# Autodesk Inventor assembly: Skateboard Remote
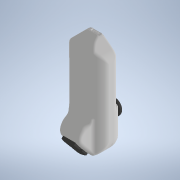
[picture p0: Inventor's stored thumbnail of the model, 180x180]
Saved by Autodesk Inventor 2020 (Build 240168000, 168)
## iProperties
Created: 2021-01-14
Part Number: Skateboard Remote
Document SubType Name: Assembly
Designer: Luke
Author: Luke
## Documents named in this file (19)
- C:\Users\Luke\Documents\Git Projects\Electric Skateboard V2\Part Files\Remote Parts\Skateboard Remote.iam
- C:\Users\Luke\Documents\Git Projects\Electric Skateboard V2\Part Files\Remote Parts\PCB.ipt
- C:\Users\Luke\Documents\Git Projects\Electric Skateboard V2\Part Files\Remote Parts\Battery Spacer.ipt
- C:\Users\Luke\Documents\Git Projects\Electric Skateboard V2\Part Files\Remote Parts\Battery.ipt
- C:\Users\Luke\Documents\Git Projects\Electric Skateboard V2\Part Files\Remote Parts\Button Module.ipt
- C:\Users\Luke\Documents\Git Projects\Electric Skateboard V2\Part Files\Remote Parts\Joystick.ipt
- C:\Users\Luke\Documents\Git Projects\Electric Skateboard V2\Part Files\Remote Parts\Button.ipt
- C:\Users\Luke\Documents\Git Projects\Electric Skateboard V2\Part Files\Remote Parts\Joystick Cap.ipt
- C:\Users\Luke\Documents\Git Projects\Electric Skateboard V2\Part Files\Remote Parts\Display.ipt
- C:\Users\Luke\Documents\Git Projects\Electric Skateboard V2\Part Files\Remote Parts\Vibrator Motor.ipt
- C:\Users\Luke\Documents\Git Projects\Electric Skateboard V2\Part Files\Remote Parts\USB Port.ipt
- C:\Users\Luke\Documents\Git Projects\Electric Skateboard V2\Part Files\Remote Parts\BMS.ipt
- C:\Users\Luke\Documents\Git Projects\Electric Skateboard V2\Part Files\Remote Parts\Finger Button.ipt
- C:\Users\Luke\Documents\Git Projects\Electric Skateboard V2\Part Files\Remote Parts\Enclosure Bottom Slim.ipt
- C:\Users\Luke\Documents\Git Projects\Electric Skateboard V2\Part Files\Remote Parts\Power Swicth.ipt
- C:\Users\Luke\Documents\Git Projects\Electric Skateboard V2\Part Files\Remote Parts\Button Holder Bottom.ipt
- C:\Users\Luke\Documents\Git Projects\Electric Skateboard V2\Part Files\Remote Parts\Button Holder Top.ipt
- C:\Users\Luke\Documents\Git Projects\Electric Skateboard V2\Part Files\Remote Parts\Enclosure Top.ipt
- C:\Users\Luke\Documents\Git Projects\Electric Skateboard V2\Part Files\Remote Parts\Power Switch Cap.ipt
## Components (21 placed, 18 different names)
1. PCB:1 — Mate:1, Flush:1, Flush:2, Mate:2, Flush:6, Flush:8, Flush:9, Flush:10, Flush:12, Mate:27, Mate:28, Mate:29, Mate:30, Flush:15, Mate:31, Mate:32, Flush:16, Flush:30, Flush:32, Flush:33, Mate:59, Mate:60, Flush:34, Mate:61, Mate:62, Mate:63, Mate:64, Mate:72, Mate:73, Flush:76
2. Display:1 — Mate:72, Mate:73, Flush:76
3. Battery Spacer:1 — Mate:1, Flush:1, Flush:2, Flush:3
4. Battery:1 — Flush:3, Mate:2, Flush:12
5. Joystick:1 — Flush:6, Flush:8, Flush:9, Flush:10, Mate:69, Mate:70
6. Joystick Cap:1 — Mate:69, Mate:70
7. Power Swicth:1 — Mate:60, Flush:34, Mate:61, Mate:74, Mate:75, Flush:77
8. Power Switch Cap:1 — Mate:74, Mate:75, Flush:77
9. Vibrator Motor:1 — Mate:27, Mate:28, Mate:29
10. USB Port:1 — Mate:30, Flush:15, Mate:31
11. BMS:1 — Mate:32, Flush:16, Mate:33, Flush:17, Mate:34, Flush:30
12. USB Port:2 — Mate:33, Flush:17, Mate:34
13. Button Holder Top:1 — Mate:62, Mate:63, Mate:64, Flush:36
14. Button Holder Bottom:1 — Flush:36, Flush:68, Mate:67, Mate:68
15. Button Module:1 — Mate:6, Mate:7, Mate:8, Mate:9, Mate:10, Mate:11, Flush:68, Mate:67, Mate:68
16. Button:3 — Mate:9, Mate:10, Mate:11, Mate:54, Mate:56, Mate:58
17. Button:2 — Mate:6, Mate:7, Mate:8, Mate:55, Flush:29, Mate:57
18. Finger Button:2 — Mate:54, Mate:56, Mate:58, Flush:69, Flush:70
19. Finger Button:1 — Mate:55, Flush:29, Mate:57
20. Enclosure Bottom Slim:1 — Flush:32, Flush:33, Mate:59, Flush:69, Flush:70, Flush:78, Flush:79, Mate:76
21. Enclosure Top:1 — Flush:78, Flush:79, Mate:76
## Relationships (60: Mate 36, Flush 24)
- Mate:1: PCB:1 ↔ Battery Spacer:1
- Flush:1 (9.27 mm): PCB:1 ↔ Battery Spacer:1
- Flush:2 (6.4 mm): PCB:1 ↔ Battery Spacer:1
- Flush:3: Battery Spacer:1 ↔ Battery:1
- Mate:2: PCB:1 ↔ Battery:1
- Flush:6: PCB:1 ↔ Joystick:1
- Flush:8: PCB:1 ↔ Joystick:1
- Flush:9: PCB:1 ↔ Joystick:1
- Flush:10: PCB:1 ↔ Joystick:1
- Mate:6: Button Module:1 ↔ Button:2
- Mate:7: Button Module:1 ↔ Button:2
- Mate:8: Button Module:1 ↔ Button:2
- Mate:9: Button Module:1 ↔ Button:3
- Mate:10: Button Module:1 ↔ Button:3
- Mate:11: Button Module:1 ↔ Button:3
- Flush:12 (5 mm): PCB:1 ↔ Battery:1
- Mate:27: PCB:1 ↔ Vibrator Motor:1
- Mate:28 (-10 mm): PCB:1 ↔ Vibrator Motor:1
- Mate:29 (-15 mm): PCB:1 ↔ Vibrator Motor:1
- Mate:30: PCB:1 ↔ USB Port:1
- Flush:15: PCB:1 ↔ USB Port:1
- Mate:31: PCB:1 ↔ USB Port:1
- Mate:32: PCB:1 ↔ BMS:1
- Flush:16: PCB:1 ↔ BMS:1
- Mate:33: BMS:1 ↔ USB Port:2
- Flush:17: BMS:1 ↔ USB Port:2
- Mate:34: BMS:1 ↔ USB Port:2
- Mate:54: Button:3 ↔ Finger Button:2
- Mate:55: Button:2 ↔ Finger Button:1
- Mate:56: Button:3 ↔ Finger Button:2
- Flush:29: Button:2 ↔ Finger Button:1
- Mate:57: Button:2 ↔ Finger Button:1
- Mate:58: Button:3 ↔ Finger Button:2
- Flush:30 (8.38 mm): PCB:1 ↔ BMS:1
- Flush:32: PCB:1 ↔ Enclosure Bottom Slim:1
- Flush:33: PCB:1 ↔ Enclosure Bottom Slim:1
- Mate:59: PCB:1 ↔ Enclosure Bottom Slim:1
- Mate:60: PCB:1 ↔ Power Swicth:1
- Flush:34: PCB:1 ↔ Power Swicth:1
- Mate:61: PCB:1 ↔ Power Swicth:1
- Mate:62: PCB:1 ↔ Button Holder Top:1
- Mate:63: PCB:1 ↔ Button Holder Top:1
- Mate:64: PCB:1 ↔ Button Holder Top:1
- Flush:36: Button Holder Top:1 ↔ Button Holder Bottom:1
- Flush:68: Button Holder Bottom:1 ↔ Button Module:1
- Mate:67: Button Holder Bottom:1 ↔ Button Module:1
- Mate:68: Button Holder Bottom:1 ↔ Button Module:1
- Flush:69: Finger Button:2 ↔ Enclosure Bottom Slim:1
- Flush:70 (0.15 mm): Finger Button:2 ↔ Enclosure Bottom Slim:1
- Mate:69 (2.75 mm): Joystick:1 ↔ Joystick Cap:1
- Mate:70: Joystick:1 ↔ Joystick Cap:1
- Mate:72: PCB:1 ↔ Display:1
- Mate:73: PCB:1 ↔ Display:1
- Flush:76 (-35.76 mm): PCB:1 ↔ Display:1
- Mate:74: Power Swicth:1 ↔ Power Switch Cap:1
- Mate:75: Power Swicth:1 ↔ Power Switch Cap:1
- Flush:77: Power Swicth:1 ↔ Power Switch Cap:1
- Flush:78: Enclosure Bottom Slim:1 ↔ Enclosure Top:1
- Flush:79: Enclosure Bottom Slim:1 ↔ Enclosure Top:1
- Mate:76: Enclosure Bottom Slim:1 ↔ Enclosure Top:1
